# Autodesk Inventor assembly: Assembly1
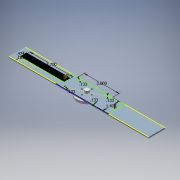
[picture p0: Inventor's stored thumbnail of the model, 180x180]
Saved by Autodesk Inventor 2016 (Build 200138000, 138)
## iProperties
Created: 2017-12-11
Part Number: Assembly1
Document SubType Name: Assembly
Designer: student
Author: student
## Documents named in this file (3)
- C:\Users\student\Documents\GitHub\POV2017\INVENTOR\Assembly1.iam
- C:\Users\student\Documents\GitHub\POV2017\INVENTOR\Base.ipt
- C:\Users\student\Documents\GitHub\POV2017\INVENTOR\Shaft.ipt
## Components (2 placed, 2 different names)
1. Base:1 — Mate:2, Mate:3, Mate:4
2. Shaft:1 — Mate:2, Mate:3, Mate:4
## Relationships (3: Mate 3)
- Mate:2: Base:1 ↔ Shaft:1
- Mate:3: Base:1 ↔ Shaft:1
- Mate:4: Base:1 ↔ Shaft:1
